# Autodesk Inventor assembly: ASSEMBLY_piston_connecting_rod
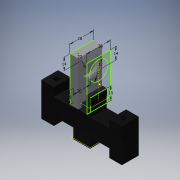
[picture p0: Inventor's stored thumbnail of the model, 180x180]
Saved by Autodesk Inventor 2018 (Build 220112000, 112)
## iProperties
Created: 2026-07-08
Part Number: ASSEMBLY_piston_connecting_rod
Document SubType Name: Assembly
Designer: neo
Author: neo
## Documents named in this file (3)
- C:\Users\neo\Documents\neoatlantis-shared\projects\kreion\design2\ASSEMBLY_piston_connecting_rod.iam
- C:\Users\neo\Documents\neoatlantis-shared\projects\kreion\design2\PRING_piston.ipt
- C:\Users\neo\Documents\neoatlantis-shared\projects\kreion\design2\PISTON_bearing.ipt
## Components (3 placed, 2 different names)
1. PRING_piston:1 — Mate:2, Mate:3, Mate:4
2. PISTON_bearing:1 — Mate:1, Flush:1, Flush:2, Mate:2, Mate:3, Mate:4
3. PISTON_bearing:2 — Mate:1, Flush:1, Flush:2
## Relationships (6: Mate 4, Flush 2)
- Mate:1: PISTON_bearing:1 ↔ PISTON_bearing:2
- Flush:1: PISTON_bearing:1 ↔ PISTON_bearing:2
- Flush:2: PISTON_bearing:1 ↔ PISTON_bearing:2
- Mate:2: PRING_piston:1 ↔ PISTON_bearing:1
- Mate:3: PRING_piston:1 ↔ PISTON_bearing:1
- Mate:4: PRING_piston:1 ↔ PISTON_bearing:1
